# Autodesk Inventor assembly: AdjusterAssembly_2019
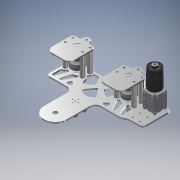
[picture p0: Inventor's stored thumbnail of the model, 180x180]
Saved by Autodesk Inventor 2019.4 (Build 234330000, 330)
## iProperties
Created: 2020-02-06
Part Number: AdjusterAssembly_2019
Document SubType Name: Assembly
Designer: Paul Lefeuvre
Mass: 1470.23 g
Surface Area: 3224.18 cm^2
Volume: 760.064 cm^3
Density: 1.93436 g/cm^3
Author: Paul Lefeuvre
## Documents named in this file (12)
- C:\Users\admin\Desktop\FRC 2020 Engineering\GitHub\7738-2020\7738-Adjuster\AdjusterAssembly_2019.iam
- C:\Users\admin\Desktop\FRC 2020 Engineering\GitHub\7738-2020\7738-Adjuster\MainHolder2_2019.ipt
- C:\Users\admin\Desktop\FRC 2020 Engineering\GitHub\7738-2020\7738-Adjuster\Mini V Gantry Kit.iam
- C:\Users\admin\Desktop\FRC 2020 Engineering\GitHub\7738-2020\7738-Adjuster\Colson_Performa_1_625_x_0_875_1_2_Hex_bore_217-4045.ipt
- C:\Users\admin\Desktop\FRC 2020 Engineering\GitHub\7738-2020\7738-Adjuster\Spacer1_2019.ipt
- C:\Users\admin\Desktop\FRC 2020 Engineering\GitHub\7738-2020\7738-Adjuster\CaseSheet_2019.ipt
- C:\Users\admin\Desktop\FRC 2020 Engineering\GitHub\7738-2020\7738-Adjuster\F6801_2019.ipt
- C:\Users\admin\Desktop\FRC 2020 Engineering\GitHub\7738-2020\7738-Adjuster\F6800_2019.ipt
- C:\Users\admin\Desktop\FRC 2020 Engineering\GitHub\7738-2020\7738-Adjuster\Axle1_2019.ipt
- C:\Users\admin\Desktop\FRC 2020 Engineering\GitHub\7738-2020\7738-Adjuster\Axle2_2019.ipt
- C:\Users\admin\Desktop\FRC 2020 Engineering\GitHub\7738-2020\7738-Adjuster\775pro_217-4347.ipt
- C:\Users\admin\Desktop\FRC 2020 Engineering\GitHub\7738-2020\7738-Adjuster\2 Stage SD - 57 Sport.ipt
## Components (26 placed, 11 different names)
1. MainHolder2_2019:1 — Flush:1, Insert:28, Insert:29, Insert:30, Insert:31, Insert:32, Insert:33, Mate:2, Insert:34, Insert:35, Insert:36, Insert:37, Insert:38, Insert:39, Insert:40, Insert:41, Mate:3
2. Mini V Gantry Kit:1 [sub-assembly] — Insert:28, Insert:29
3. Spacer1_2019:1 — Insert:10, Insert:33
4. Spacer1_2019:2 — Insert:13, Insert:32
5. Spacer1_2019:3 — Insert:17, Insert:39
6. Spacer1_2019:4 — Insert:15, Insert:37
7. Spacer1_2019:5 — Insert:16, Insert:38
8. Spacer1_2019:6 — Insert:11, Insert:31
9. Spacer1_2019:7 — Insert:14, Insert:35
10. Spacer1_2019:8 — Insert:12, Insert:34
11. CaseSheet_2019:1 — Insert:10, Insert:11, Insert:12, Insert:13, Insert:18
12. CaseSheet_2019:2 — Insert:14, Insert:15, Insert:16, Insert:17, Insert:19
13. F6801_2019:1 — Insert:22, Insert:41
14. F6801_2019:2 — Insert:23, Insert:40
15. F6800_2019:1 — Insert:18
16. F6800_2019:2 — Insert:19
17. Axle1_2019:1 — Insert:23, Insert:24, Angle:2, Insert:25, Angle:3
18. Axle2_2019:1 — Insert:22, Insert:26, Angle:4, Insert:27, Angle:5
19. Colson_Performa_1_625_x_0_875_1_2_Hex_bore_217-4045:1 — Insert:24, Angle:2
20. Colson_Performa_1_625_x_0_875_1_2_Hex_bore_217-4045:2 — Insert:26, Angle:4
21. Colson_Performa_1_625_x_0_875_1_2_Hex_bore_217-4045:3 — Insert:27, Angle:5
22. Colson_Performa_1_625_x_0_875_1_2_Hex_bore_217-4045:4 — Insert:25, Angle:3
23. Spacer1_2019:9 — Insert:36
24. Spacer1_2019:10 — Insert:30
25. 775pro_217-4347:1 — Insert:58, Insert:59
26. 2 Stage SD - 57 Sport:1 — Insert:58, Insert:59
## Relationships (39: Insert 32, Angle 4, Mate 2, Flush 1)
- Insert:10 (1 mm): Spacer1_2019:1 ↔ CaseSheet_2019:1
- Insert:11 (1 mm): Spacer1_2019:6 ↔ CaseSheet_2019:1
- Insert:12 (1 mm): Spacer1_2019:8 ↔ CaseSheet_2019:1
- Insert:13 (1 mm): Spacer1_2019:2 ↔ CaseSheet_2019:1
- Insert:14 (1 mm): Spacer1_2019:7 ↔ CaseSheet_2019:2
- Insert:15 (1 mm): Spacer1_2019:4 ↔ CaseSheet_2019:2
- Insert:16 (1 mm): Spacer1_2019:5 ↔ CaseSheet_2019:2
- Insert:17 (1 mm): Spacer1_2019:3 ↔ CaseSheet_2019:2
- Insert:18 (0.6 mm): CaseSheet_2019:1 ↔ F6800_2019:1
- Insert:19 (0.6 mm): CaseSheet_2019:2 ↔ F6800_2019:2
- Insert:22 (0.6 mm): F6801_2019:1 ↔ Axle2_2019:1
- Insert:23 (0.6 mm): F6801_2019:2 ↔ Axle1_2019:1
- Insert:24 (0.6 mm): Axle1_2019:1 ↔ Colson_Performa_1_625_x_0_875_1_2_Hex_bore_217-4045:1
- Angle:2 (0 deg): Axle1_2019:1 ↔ Colson_Performa_1_625_x_0_875_1_2_Hex_bore_217-4045:1
- Insert:25 (0.6 mm): Axle1_2019:1 ↔ Colson_Performa_1_625_x_0_875_1_2_Hex_bore_217-4045:4
- Angle:3 (0 deg): Axle1_2019:1 ↔ Colson_Performa_1_625_x_0_875_1_2_Hex_bore_217-4045:4
- Insert:26 (0.3 mm): Axle2_2019:1 ↔ Colson_Performa_1_625_x_0_875_1_2_Hex_bore_217-4045:2
- Angle:4 (0 deg): Axle2_2019:1 ↔ Colson_Performa_1_625_x_0_875_1_2_Hex_bore_217-4045:2
- Insert:27 (0.3 mm): Axle2_2019:1 ↔ Colson_Performa_1_625_x_0_875_1_2_Hex_bore_217-4045:3
- Angle:5 (0 deg): Axle2_2019:1 ↔ Colson_Performa_1_625_x_0_875_1_2_Hex_bore_217-4045:3
- Flush:1 (-199.031 mm): MainHolder2_2019:1
- Insert:28 (0.6 mm): MainHolder2_2019:1 ↔ Mini V Gantry Kit:1
- Insert:29 (0.6 mm): MainHolder2_2019:1 ↔ Mini V Gantry Kit:1
- Insert:30 (1 mm): MainHolder2_2019:1 ↔ Spacer1_2019:10
- Insert:31 (1 mm): MainHolder2_2019:1 ↔ Spacer1_2019:6
- Insert:32 (1 mm): MainHolder2_2019:1 ↔ Spacer1_2019:2
- Insert:33 (1 mm): MainHolder2_2019:1 ↔ Spacer1_2019:1
- Mate:2: MainHolder2_2019:1
- Insert:34 (1 mm): MainHolder2_2019:1 ↔ Spacer1_2019:8
- Insert:35 (1 mm): MainHolder2_2019:1 ↔ Spacer1_2019:7
- Insert:36 (1 mm): MainHolder2_2019:1 ↔ Spacer1_2019:9
- Insert:37 (1 mm): MainHolder2_2019:1 ↔ Spacer1_2019:4
- Insert:38 (1 mm): MainHolder2_2019:1 ↔ Spacer1_2019:5
- Insert:39 (1 mm): MainHolder2_2019:1 ↔ Spacer1_2019:3
- Insert:40 (0.6 mm): MainHolder2_2019:1 ↔ F6801_2019:2
- Insert:41 (0.6 mm): MainHolder2_2019:1 ↔ F6801_2019:1
- Mate:3: MainHolder2_2019:1
- Insert:58 (0.6 mm): 775pro_217-4347:1 ↔ 2 Stage SD - 57 Sport:1
- Insert:59 (0.6 mm): 775pro_217-4347:1 ↔ 2 Stage SD - 57 Sport:1
